# Autodesk Inventor assembly: 2617488 EAMM-U-70-D40-60P-96
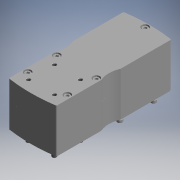
[picture p0: Inventor's stored thumbnail of the model, 180x180]
Saved by Autodesk Inventor 2017.3 (Build 213256000, 256)
## iProperties
Category: PARTsolutions
Company: FESTO
Part Number: 2617488 EAMM-U-70-D40-60P-96
Catalog Web Link: www.cadenas.de
Description: EAMM-U-parallel kit
Vendor: FESTO
Document SubType Name: Assembly
Designer: partserver
Manufacturer: FESTO
Mass: 1730 g
Surface Area: 1149.62 cm^2
Volume: 401.327 cm^3
Density: 4.3107 g/cm^3
Title: 2617488 EAMM-U-70-D40-60P-96
Author: Cadenas PARTsolutions
Comments: parallel kit
PSOL_IDENT_0: {ATYP=ASSISTANT},{DATA=script=$CADENAS_DATA/23d-libs/festo/webfesto.vbb&M_FAMILY=EAMM&M_GROUP=01&M_P
PSOL_IDENT_1: ARTNO=2617488&IDCODE1=EAMM-U-70-D40-60P-96&IDCODE2=&customer_number_cns=&MATES=1&LOD=HI&LOCKERP=0&SI
PSOL_IDENT_2: NGLEPART=1}
NB: 2617488 EAMM-U-70-D40-60P-96
NN: EAMM-U
NT: parallel kit
NBSYN: $TNR. $TYP.
LINA: 2617488 EAMM-U-70-D40-60P-96
CATALOG: Festo
TNR: 2617488
TYP: EAMM-U-70-D40-60P-96
B1: 70
B2: 0
B3: 38
B4: 0
B5: 38
B6: 58
D1: 50.5
D2: 70
D3: 40
D4: 5.300
D5: 6.6
D6: M6
D7: 0
H1: 173.5
H2: 0
H3: 38
H4: 0
H5: 38
H6: 34.5
H7: 96
H8: 10
H9: 32.5
H10: 100.5
H11: 0
H12: 2
L1: 64.5
L2: 0
L3: 0
L4: 0
T1: 15
W1: 45
W2: 0
CNSMASSEXACT: 1.73
SUPPLIER: FESTO
ARTICLENO: 2617488 EAMM-U-70-D40-60P-96
BOMINFO: 2617488 EAMM-U-70-D40-60P-96
CREATOR: CADENAS GmbH
## Documents named in this file (7)
- e:\temp\worker_11\temp\exporttempdir_6360_28_xBRU0\format_0\2617488 EAMM-U-70-D40-60P-96.iam
- e:\temp\worker_11\temp\exporttempdir_6360_28_xBRU0\format_0\2607475 EAMM-U-70-D40-60P-96---(UT).ipt
- e:\temp\worker_11\temp\exporttempdir_6360_28_xBRU0\format_0\2610112 EAMM-U-70-D40-___-173---(OT).ipt
- e:\temp\worker_11\temp\exporttempdir_6360_28_xBRU0\format_0\DIN-912 - M5x35(F).ipt
- e:\temp\worker_11\temp\exporttempdir_6360_28_xBRU0\format_0\DIN 557 - M4.ipt
- e:\temp\worker_11\temp\exporttempdir_6360_28_xBRU0\format_0\DIN-6912 - M6x18(F).ipt
- e:\temp\worker_11\temp\exporttempdir_6360_28_xBRU0\format_0\DIN-912 - M4x16(F).ipt
## Components (19 placed, 6 different names)
1. 2607475 EAMM-U-70-D40-60P-96---(UT):1 — AS_1_XY@1 <-> MONTAGE_XY@12, AS_1_Z@1 <-> MONTAGE_Z@12, AS_1_YZ@1 <-> MONTAGE_YZ@12, AS_2_XY@1 <-> MONTAGE_XY@13, AS_2_Z@1 <-> MONTAGE_Z@13, AS_2_YZ@1 <-> MONTAGE_YZ@13, AS_3_XY@1 <-> MONTAGE_XY@14, AS_3_Z@1 <-> MONTAGE_Z@14, AS_3_YZ@1 <-> MONTAGE_YZ@14, AS_4_XY@1 <-> MONTAGE_XY@15, AS_4_Z@1 <-> MONTAGE_Z@15, AS_4_YZ@1 <-> MONTAGE_YZ@15, MS_1_XY@1 <-> ANBAU_XY@16, MS_1_Z@1 <-> ANBAU_Z@16, MS_1_YZ@1 <-> ANBAU_YZ@16, MS_2_XY@1 <-> ANBAU_XY@17, MS_2_Z@1 <-> ANBAU_Z@17, MS_2_YZ@1 <-> ANBAU_YZ@17, MS_3_XY@1 <-> ANBAU_XY@18, MS_3_Z@1 <-> ANBAU_Z@18, MS_3_YZ@1 <-> ANBAU_YZ@18, MS_4_XY@1 <-> ANBAU_XY@19, MS_4_Z@1 <-> ANBAU_Z@19, MS_4_YZ@1 <-> ANBAU_YZ@19
2. 2610112 EAMM-U-70-D40-___-173---(OT):1
3. DIN-912 - M5x35(F):1
4. DIN-912 - M5x35(F):2
5. DIN-912 - M5x35(F):3
6. DIN-912 - M5x35(F):4
7. DIN-912 - M5x35(F):5
8. DIN 557 - M4:1
9. DIN 557 - M4:2
10. DIN 557 - M4:3
11. DIN 557 - M4:4
12. DIN-6912 - M6x18(F):1 — AS_1_XY@1 <-> MONTAGE_XY@12, AS_1_Z@1 <-> MONTAGE_Z@12, AS_1_YZ@1 <-> MONTAGE_YZ@12
13. DIN-6912 - M6x18(F):2 — AS_2_XY@1 <-> MONTAGE_XY@13, AS_2_Z@1 <-> MONTAGE_Z@13, AS_2_YZ@1 <-> MONTAGE_YZ@13
14. DIN-6912 - M6x18(F):3 — AS_3_XY@1 <-> MONTAGE_XY@14, AS_3_Z@1 <-> MONTAGE_Z@14, AS_3_YZ@1 <-> MONTAGE_YZ@14
15. DIN-6912 - M6x18(F):4 — AS_4_XY@1 <-> MONTAGE_XY@15, AS_4_Z@1 <-> MONTAGE_Z@15, AS_4_YZ@1 <-> MONTAGE_YZ@15
16. DIN-912 - M4x16(F):1 — MS_1_XY@1 <-> ANBAU_XY@16, MS_1_Z@1 <-> ANBAU_Z@16, MS_1_YZ@1 <-> ANBAU_YZ@16
17. DIN-912 - M4x16(F):2 — MS_2_XY@1 <-> ANBAU_XY@17, MS_2_Z@1 <-> ANBAU_Z@17, MS_2_YZ@1 <-> ANBAU_YZ@17
18. DIN-912 - M4x16(F):3 — MS_3_XY@1 <-> ANBAU_XY@18, MS_3_Z@1 <-> ANBAU_Z@18, MS_3_YZ@1 <-> ANBAU_YZ@18
19. DIN-912 - M4x16(F):4 — MS_4_XY@1 <-> ANBAU_XY@19, MS_4_Z@1 <-> ANBAU_Z@19, MS_4_YZ@1 <-> ANBAU_YZ@19
## Relationships (24: Mate 16, Angle 8)
- AS_1_XY@1 <-> MONTAGE_XY@12 [Mate]: 2607475 EAMM-U-70-D40-60P-96---(UT):1 ↔ DIN-6912 - M6x18(F):1
- AS_1_Z@1 <-> MONTAGE_Z@12 [Mate]: 2607475 EAMM-U-70-D40-60P-96---(UT):1 ↔ DIN-6912 - M6x18(F):1
- AS_1_YZ@1 <-> MONTAGE_YZ@12 [Angle] (0 deg): 2607475 EAMM-U-70-D40-60P-96---(UT):1 ↔ DIN-6912 - M6x18(F):1
- AS_2_XY@1 <-> MONTAGE_XY@13 [Mate]: 2607475 EAMM-U-70-D40-60P-96---(UT):1 ↔ DIN-6912 - M6x18(F):2
- AS_2_Z@1 <-> MONTAGE_Z@13 [Mate]: 2607475 EAMM-U-70-D40-60P-96---(UT):1 ↔ DIN-6912 - M6x18(F):2
- AS_2_YZ@1 <-> MONTAGE_YZ@13 [Angle] (0 deg): 2607475 EAMM-U-70-D40-60P-96---(UT):1 ↔ DIN-6912 - M6x18(F):2
- AS_3_XY@1 <-> MONTAGE_XY@14 [Mate]: 2607475 EAMM-U-70-D40-60P-96---(UT):1 ↔ DIN-6912 - M6x18(F):3
- AS_3_Z@1 <-> MONTAGE_Z@14 [Mate]: 2607475 EAMM-U-70-D40-60P-96---(UT):1 ↔ DIN-6912 - M6x18(F):3
- AS_3_YZ@1 <-> MONTAGE_YZ@14 [Angle] (0 deg): 2607475 EAMM-U-70-D40-60P-96---(UT):1 ↔ DIN-6912 - M6x18(F):3
- AS_4_XY@1 <-> MONTAGE_XY@15 [Mate]: 2607475 EAMM-U-70-D40-60P-96---(UT):1 ↔ DIN-6912 - M6x18(F):4
- AS_4_Z@1 <-> MONTAGE_Z@15 [Mate]: 2607475 EAMM-U-70-D40-60P-96---(UT):1 ↔ DIN-6912 - M6x18(F):4
- AS_4_YZ@1 <-> MONTAGE_YZ@15 [Angle] (0 deg): 2607475 EAMM-U-70-D40-60P-96---(UT):1 ↔ DIN-6912 - M6x18(F):4
- MS_1_XY@1 <-> ANBAU_XY@16 [Mate]: 2607475 EAMM-U-70-D40-60P-96---(UT):1 ↔ DIN-912 - M4x16(F):1
- MS_1_Z@1 <-> ANBAU_Z@16 [Mate]: 2607475 EAMM-U-70-D40-60P-96---(UT):1 ↔ DIN-912 - M4x16(F):1
- MS_1_YZ@1 <-> ANBAU_YZ@16 [Angle] (0 deg): 2607475 EAMM-U-70-D40-60P-96---(UT):1 ↔ DIN-912 - M4x16(F):1
- MS_2_XY@1 <-> ANBAU_XY@17 [Mate]: 2607475 EAMM-U-70-D40-60P-96---(UT):1 ↔ DIN-912 - M4x16(F):2
- MS_2_Z@1 <-> ANBAU_Z@17 [Mate]: 2607475 EAMM-U-70-D40-60P-96---(UT):1 ↔ DIN-912 - M4x16(F):2
- MS_2_YZ@1 <-> ANBAU_YZ@17 [Angle] (0 deg): 2607475 EAMM-U-70-D40-60P-96---(UT):1 ↔ DIN-912 - M4x16(F):2
- MS_3_XY@1 <-> ANBAU_XY@18 [Mate]: 2607475 EAMM-U-70-D40-60P-96---(UT):1 ↔ DIN-912 - M4x16(F):3
- MS_3_Z@1 <-> ANBAU_Z@18 [Mate]: 2607475 EAMM-U-70-D40-60P-96---(UT):1 ↔ DIN-912 - M4x16(F):3
- MS_3_YZ@1 <-> ANBAU_YZ@18 [Angle] (0 deg): 2607475 EAMM-U-70-D40-60P-96---(UT):1 ↔ DIN-912 - M4x16(F):3
- MS_4_XY@1 <-> ANBAU_XY@19 [Mate]: 2607475 EAMM-U-70-D40-60P-96---(UT):1 ↔ DIN-912 - M4x16(F):4
- MS_4_Z@1 <-> ANBAU_Z@19 [Mate]: 2607475 EAMM-U-70-D40-60P-96---(UT):1 ↔ DIN-912 - M4x16(F):4
- MS_4_YZ@1 <-> ANBAU_YZ@19 [Angle] (0 deg): 2607475 EAMM-U-70-D40-60P-96---(UT):1 ↔ DIN-912 - M4x16(F):4
